# Autodesk Inventor assembly: A90P
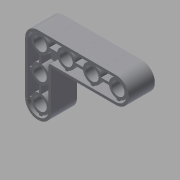
[picture p0: Inventor's stored thumbnail of the model, 180x180]
Saved by Autodesk Inventor 2019.3 (Build 233278000, 278)
## iProperties
Created: 2019-01-31
Part Number: A90P
Document SubType Name: Assembly
Designer: Varga Daniel
Vertical_hole_count: 3,000 ul
Horizontal_hole_count: 4,000 ul
Author: Varga Daniel
## Documents named in this file (9)
- C:\!_Dani\!_cloud\OneDrive\!_munka\Revolution\RevvyDemoKit\Structural parts\Beams\Angled Beams\L-V-shape beams.iam
- C:\!_Dani\!_cloud\OneDrive\!_munka\Revolution\RevvyDemoKit\Structural parts\Beams\Angled Beams\Bent beam base.ipt
- C:\!_Dani\!_cloud\OneDrive\!_munka\Revolution\RevvyDemoKit\Structural parts\Beams\beam_single_end_part.ipt
- C:\!_Dani\!_cloud\OneDrive\!_munka\Revolution\RevvyDemoKit\Structural parts\Beams\beam_single_inner_part.ipt
- C:\!_Dani\!_cloud\OneDrive\!_munka\Revolution\RevvyDemoKit\Structural parts\Beams\Angled Beams\Bent beam base\Bent beam base-90.ipt
- A120.iam
- A135.iam
- A90L.iam
- A90P.iam
## Components (6 placed, 3 different names)
1. Bent beam base-90:1 — Flush:1, Flush:2, Flush:3, Flush:4, Mate:1, Mate:2, Flush:5, Flush:6, Mate:3, Flush:7, Flush:8, Mate:4
2. beam_single_end_part:1 — Flush:3, Flush:4, Mate:1
3. beam_single_end_part:2 — Flush:5, Flush:6, Mate:3
4. beam_single_inner_part:2 — Flush:1, Flush:2, Mate:2
5. beam_single_inner_part:3
6. beam_single_inner_part:1 — Flush:7, Flush:8, Mate:4
## Component patterns: (2 elements, first: beam_single_inner_part:2), (1 elements, first: beam_single_inner_part:1)
## Relationships (12: Flush 8, Mate 4)
- Flush:1: Bent beam base-90:1 ↔ beam_single_inner_part:2
- Flush:2: Bent beam base-90:1 ↔ beam_single_inner_part:2
- Flush:3: Bent beam base-90:1 ↔ beam_single_end_part:1
- Flush:4: Bent beam base-90:1 ↔ beam_single_end_part:1
- Mate:1 (20 mm): Bent beam base-90:1 ↔ beam_single_end_part:1
- Mate:2: Bent beam base-90:1 ↔ beam_single_inner_part:2
- Flush:5: Bent beam base-90:1 ↔ beam_single_end_part:2
- Flush:6: Bent beam base-90:1 ↔ beam_single_end_part:2
- Mate:3 (10 mm): Bent beam base-90:1 ↔ beam_single_end_part:2
- Flush:7: Bent beam base-90:1 ↔ beam_single_inner_part:1
- Flush:8: Bent beam base-90:1 ↔ beam_single_inner_part:1
- Mate:4: Bent beam base-90:1 ↔ beam_single_inner_part:1
